# Autodesk Inventor assembly: TinyTurner
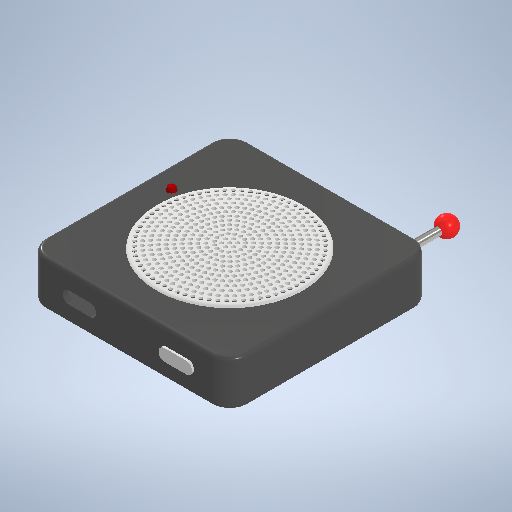
[picture p0: Inventor's stored thumbnail of the model, 512x512]
Saved by Autodesk Inventor 2026 (Build 300175050, 175E)
## iProperties
Created: 2025-07-10
Part Number: TinyTurner
Document SubType Name: Assembly
Designer: Jochen Alt
Author: Jochen Alt
## Documents named in this file (6)
- D:\Projects\TinyTurner\CAD\TinyTurner.iam
- D:\Projects\TinyTurner\CAD\Box.ipt
- D:\Projects\TinyTurner\CAD\Antenna.ipt
- D:\Projects\TinyTurner\CAD\Grid.ipt
- D:\Projects\TinyTurner\CAD\External Components\led-2mm\Led_2mm\Led_2mm\Led_2mm.ipt
- D:\Projects\TinyTurner\CAD\Button Cap.ipt
## Components (5 placed, 5 different names)
1. Box:1 — Mate:1, Mate:2, Mate:3, Mate:4, Mate:5, Mate:6, Angle:1, Mate:7
2. Antenna:1 — Mate:1
3. Grid:1 — Mate:2, Mate:3
4. Led_2mm:1 — Mate:4, Mate:5
5. Button Cap:1 — Mate:6, Angle:1, Mate:7
## Relationships (8: Mate 7, Angle 1)
- Mate:1: Box:1 ↔ Antenna:1
- Mate:2: Box:1 ↔ Grid:1
- Mate:3: Box:1 ↔ Grid:1
- Mate:4: Box:1 ↔ Led_2mm:1
- Mate:5: Box:1 ↔ Led_2mm:1
- Mate:6: Box:1 ↔ Button Cap:1
- Angle:1 (0 deg): Box:1 ↔ Button Cap:1
- Mate:7: Box:1 ↔ Button Cap:1
